# Autodesk Inventor assembly: sensorboard_assembly
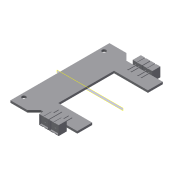
[picture p0: Inventor's stored thumbnail of the model, 180x180]
Saved by Autodesk Inventor 2014 (Build 180170000, 170)
## iProperties
Created: 2014-01-08
Part Number: sensorboard_assembly
Document SubType Name: Assembly
Designer: Felix
Author: Felix
## Documents named in this file (3)
- C:\Users\Felix\Desktop\Beep\Hardware\3D-CAD\sensorboard_assembly.iam
- C:\Users\Felix\Desktop\Beep\Hardware\3D-CAD\bottom_sensor.ipt
- C:\Users\Felix\Desktop\Beep\Hardware\3D-CAD\parts\electronic\BEEP\components\cny-70.ipt
## Components (5 placed, 2 different names)
1. bottom_sensor:1 — Passend:1, Passend:2, Passend:3, Passend:4, Passend:5, Passend:6, Passend:7, Passend:8
2. cny-70:1 — Passend:3, Passend:6, Fluchtend:2
3. cny-70:2 — Passend:4, Passend:5, Fluchtend:1
4. cny-70:3 — Passend:1, Passend:7, Fluchtend:2, Passend:9
5. cny-70:4 — Passend:2, Passend:8, Fluchtend:1, Passend:9
## Relationships (11: Mate 9, Flush 2)
- Passend:1 [Mate]: bottom_sensor:1 ↔ cny-70:3
- Passend:2 [Mate]: bottom_sensor:1 ↔ cny-70:4
- Passend:3 [Mate]: bottom_sensor:1 ↔ cny-70:1
- Passend:4 [Mate]: bottom_sensor:1 ↔ cny-70:2
- Passend:5 [Mate]: bottom_sensor:1 ↔ cny-70:2
- Passend:6 [Mate]: bottom_sensor:1 ↔ cny-70:1
- Passend:7 [Mate]: bottom_sensor:1 ↔ cny-70:3
- Passend:8 [Mate]: bottom_sensor:1 ↔ cny-70:4
- Fluchtend:1 [Flush]: cny-70:2 ↔ cny-70:4
- Fluchtend:2 [Flush]: cny-70:1 ↔ cny-70:3
- Passend:9 [Mate] (0.5 mm): cny-70:3 ↔ cny-70:4
